# Autodesk Inventor assembly: ShooterAssemblyV02
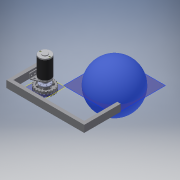
[picture p0: Inventor's stored thumbnail of the model, 180x180]
Saved by Autodesk Inventor 2016 SP1 (Build 200210100, 210)
## iProperties
Created: 2016-02-07
Part Number: ShooterAssemblyV02
Document SubType Name: Assembly
Designer: steele
Author: steele
## Documents named in this file (7)
- C:\snobotics\CAD-Development\robSteele\SnoBotics2016\2016-05-05-ShooterPrototype\ShooterAssemblyV02.iam
- C:\snobotics\CAD-Development\robSteele\SnoBotics2016\AM Parts\4 in HiGrip Wheel.iam
- C:\snobotics\CAD-Development\robSteele\SnoBotics2016\AM Parts\am-0320a_8mm_Key_Hub.ipt
- C:\snobotics\CAD-Development\robSteele\SnoBotics2016\AM Parts\MOT_CIM-Motor_217-2000.iam
- C:\snobotics\CAD-Development\robSteele\SnoBotics2016\AM Parts\AM 2488 CIM bracket.ipt
- C:\snobotics\CAD-Development\robSteele\SnoBotics2016\DraftOfBoulder.ipt
- C:\snobotics\CAD-Development\robSteele\SnoBotics2016\2016-05-05-ShooterPrototype\ShooterFrameV02.ipt
## Components (6 placed, 6 different names)
1. ShooterFrameV02:1 — Mate:4, Flush:1, Flush:2
2. 4 in HiGrip Wheel:2 [sub-assembly] — Insert:1, Mate:3
3. am-0320a_8mm_Key_Hub:1 — Insert:1, Insert:3
4. MOT_CIM-Motor_217-2000:1 [sub-assembly] — Insert:2
5. AM 2488 CIM bracket:1 — Insert:2, Insert:3, Mate:4, Flush:1, Flush:2
6. DraftOfBoulder:1 — Mate:3
## Relationships (7: Insert 3, Mate 2, Flush 2)
- Insert:1: 4 in HiGrip Wheel:2 ↔ am-0320a_8mm_Key_Hub:1
- Insert:2: MOT_CIM-Motor_217-2000:1 ↔ AM 2488 CIM bracket:1
- Insert:3: am-0320a_8mm_Key_Hub:1 ↔ AM 2488 CIM bracket:1
- Mate:3: 4 in HiGrip Wheel:2 ↔ DraftOfBoulder:1
- Mate:4: ShooterFrameV02:1 ↔ AM 2488 CIM bracket:1
- Flush:1: ShooterFrameV02:1 ↔ AM 2488 CIM bracket:1
- Flush:2: ShooterFrameV02:1 ↔ AM 2488 CIM bracket:1
